# Autodesk Inventor assembly: Full Boat
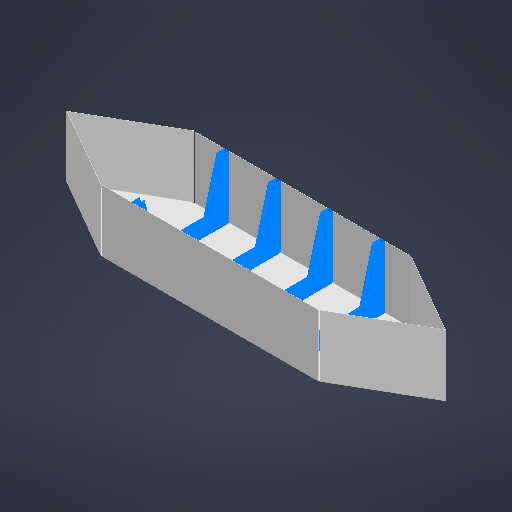
[picture p0: Inventor's stored thumbnail of the model, 512x512]
Saved by Autodesk Inventor 2025.1 (Build 291241000, 241)
## iProperties
Created: 2024-09-26
Part Number: Full Boat
Document SubType Name: Assembly
Designer: rocky
Author: rocky
## Documents named in this file (3)
- C:\Users\rocky\Documents\EDD\Boat Cad\Full Boat.iam
- C:\Users\rocky\Documents\EDD\Boat Cad\Shell.ipt
- C:\Users\rocky\Documents\EDD\Boat Cad\Div_Big.ipt
## Components (5 placed, 2 different names)
1. Shell:1 — Mate:3, Mate:7, Flush:9
2. Div_Big:1 — Flush:4, Mate:1, Flush:5, Mate:6, Flush:6, Flush:7
3. Div_Big:2 — Flush:3, Flush:4, Mate:1, Mate:2, Flush:7, Flush:8
4. Div_Big:3 — Flush:3, Mate:2, Mate:3, Flush:8, Mate:7, Flush:9
5. Div_Big:4 — Flush:5, Mate:6, Flush:6
## Relationships (12: Flush 7, Mate 5)
- Flush:3: Div_Big:2 ↔ Div_Big:3
- Flush:4: Div_Big:1 ↔ Div_Big:2
- Mate:1 (508 mm): Div_Big:1 ↔ Div_Big:2
- Mate:2 (508 mm): Div_Big:2 ↔ Div_Big:3
- Mate:3: Shell:1 ↔ Div_Big:3
- Flush:5: Div_Big:1 ↔ Div_Big:4
- Mate:6 (-508 mm): Div_Big:1 ↔ Div_Big:4
- Flush:6: Div_Big:1 ↔ Div_Big:4
- Flush:7: Div_Big:1 ↔ Div_Big:2
- Flush:8: Div_Big:2 ↔ Div_Big:3
- Mate:7: Shell:1 ↔ Div_Big:3
- Flush:9 (-254 mm): Shell:1 ↔ Div_Big:3
